# Autodesk Inventor assembly: Universal_Joint
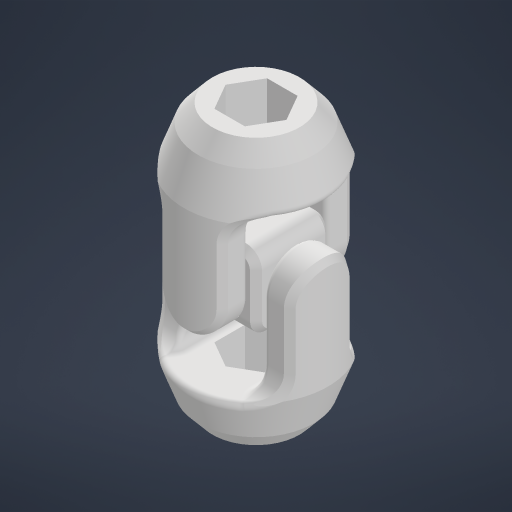
[picture p0: Inventor's stored thumbnail of the model, 512x512]
Saved by Autodesk Inventor 2024 (Build 280153000, 153)
## iProperties
Created: 2025-09-11
Part Number: Universal_Joint
Document SubType Name: Assembly
Designer: kevin
Author: kevin
## Documents named in this file (3)
- C:\Users\kevin\Desktop\SeniorDesign\Universal_Joint.iam
- C:\Users\kevin\Desktop\SeniorDesign\Universal_Joint.ipt
- C:\Users\kevin\Desktop\SeniorDesign\Universal_Joint_Connector.ipt
## Components (3 placed, 2 different names)
1. Universal_Joint:1 — Flush:1, Flush:3, Mate:1, Mate:2
2. Universal_Joint_Connector:1 — Flush:1, Flush:3
3. Universal_Joint_Connector:2 — Mate:1, Mate:2
## Relationships (4: Flush 2, Mate 2)
- Flush:1: Universal_Joint:1 ↔ Universal_Joint_Connector:1
- Flush:3 (0.3048 mm): Universal_Joint:1 ↔ Universal_Joint_Connector:1
- Mate:1: Universal_Joint:1 ↔ Universal_Joint_Connector:2
- Mate:2 (0.3 mm): Universal_Joint:1 ↔ Universal_Joint_Connector:2
